# Autodesk Inventor assembly: fakebatteryasm
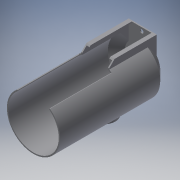
[picture p0: Inventor's stored thumbnail of the model, 180x180]
Saved by Autodesk Inventor 2018.3 (Build 223284000, 284)
## iProperties
Created: 2019-09-05
Part Number: fakebatteryasm
Document SubType Name: Assembly
Designer: Srinity
Author: Srinity
## Documents named in this file (5)
- C:\Users\Srinity\Documents\DIY Projects\NerfGun\fakebatteryasm.iam
- C:\Users\Srinity\Documents\DIY Projects\NerfGun\fakebattergasket1.ipt
- C:\Users\Srinity\Documents\DIY Projects\NerfGun\fakebattery.ipt
- C:\Users\Srinity\Documents\DIY Projects\NerfGun\fakebattergasket2.ipt
- C:\Users\Srinity\Documents\DIY Projects\NerfGun\fakebattergasket3.ipt
## Components (4 placed, 4 different names)
1. fakebattergasket1:1 — Insert:1, Angle:1, Flush:1
2. fakebattery:1 — Insert:1, Angle:1, Insert:2, Insert:3, Flush:2
3. fakebattergasket2:1 — Insert:2, Flush:1
4. fakebattergasket3:1 — Insert:3, Flush:2
## Relationships (6: Insert 3, Flush 2, Angle 1)
- Insert:1: fakebattergasket1:1 ↔ fakebattery:1
- Angle:1 (180 deg): fakebattergasket1:1 ↔ fakebattery:1
- Insert:2: fakebattery:1 ↔ fakebattergasket2:1
- Flush:1: fakebattergasket1:1 ↔ fakebattergasket2:1
- Insert:3: fakebattery:1 ↔ fakebattergasket3:1
- Flush:2: fakebattery:1 ↔ fakebattergasket3:1
